# Autodesk Inventor assembly: Center Arm Axel Attachment
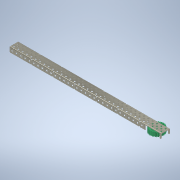
[picture p0: Inventor's stored thumbnail of the model, 180x180]
Saved by Autodesk Inventor 2020 (Build 240168000, 168)
## iProperties
Created: 2019-09-28
Part Number: Center Arm Axel Attachment
Document SubType Name: Assembly
Designer: Corey
Author: Corey
## Documents named in this file (3)
- C:\Users\Corey\Documents\Tower-Takeover-CAD\Parts\Center Arm Axel Attachment.iam
- C:\Users\Corey\Documents\Tower-Takeover-CAD\Parts\Structure\C-Channels\Aluminum\2-Wide\Aluminum C-Channel 1x2x1x35.ipt
- C:\Users\Corey\Documents\Tower-Takeover-CAD\Parts\Motion\Spur Gears\High Strength 36-tooth No Insert.iam
## Components (2 placed, 2 different names)
1. Aluminum C-Channel 1x2x1x35:1 — Mate:1, Insert:1, Insert:2
2. High Strength 36-tooth No Insert:1 [sub-assembly] — Mate:1, Insert:1, Insert:2
## Relationships (3: Insert 2, Mate 1)
- Mate:1: Aluminum C-Channel 1x2x1x35:1 ↔ High Strength 36-tooth No Insert:1
- Insert:1: Aluminum C-Channel 1x2x1x35:1 ↔ High Strength 36-tooth No Insert:1
- Insert:2: Aluminum C-Channel 1x2x1x35:1 ↔ High Strength 36-tooth No Insert:1
